# Autodesk Inventor assembly: 4in Performance Bearings
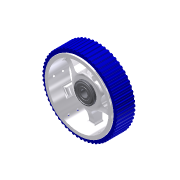
[picture p0: Inventor's stored thumbnail of the model, 180x180]
Saved by Autodesk Inventor 2011 (Build 150239000, 239)
## iProperties
Created: 2012-06-01
Part Number: 4in Performance Bearings
Document SubType Name: Assembly
Designer: Nemo
Author: Nemo
## Documents named in this file (4)
- H:\Nemo\Documents\Robotics\COTS Parts\Wheels\4in Performance Bearings nitrile.iam
- H:\Nemo\Documents\Robotics\COTS Parts\Wheels\Performance Wheel Parts\4in Performance Bearing.ipt
- H:\Nemo\Documents\Robotics\COTS Parts\Gearboxes\Bearings\Bearing 1614zz.ipt
- H:\Nemo\Documents\Robotics\COTS Parts\Wheels\Tread\Nitrile Tread.ipt
## Components (4 placed, 3 different names)
1. 4in Performance Bearing:1 — Insert:1, Insert:2, Insert:3
2. Bearing 1614zz:1 — Insert:1
3. Bearing 1614zz:2 — Insert:2
4. Nitrile Tread:1 — Insert:3
## Relationships (3: Insert 3)
- Insert:1: 4in Performance Bearing:1 ↔ Bearing 1614zz:1
- Insert:2: 4in Performance Bearing:1 ↔ Bearing 1614zz:2
- Insert:3: 4in Performance Bearing:1 ↔ Nitrile Tread:1
